# Autodesk Inventor assembly: WheelAssembly3.0
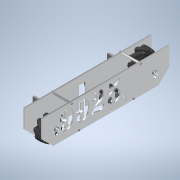
[picture p0: Inventor's stored thumbnail of the model, 180x180]
Saved by Autodesk Inventor 2021 (Build 250183000, 183)
## iProperties
Created: 2017-07-22
Part Number: WheelAssembly3.0
Document SubType Name: Assembly
Designer: User
Mass: 2301.48 g
Surface Area: 4071.67 cm^2
Volume: 902.346 cm^3
Density: 2.55055 g/cm^3
Author: User
## Documents named in this file (25)
- D:\robotics\CAD\2020-21-CAD\Drivetrain\drive train right.iam
- C:\Robotics\CAD\2016-17_CAD\Custom COTS\4inax.ipt
- C:\Robotics\CAD\2018-19_CAD\Offseason\InvertedDrivePlateOutside.ipt
- C:\Robotics\2018-19_CAD\Offseason\InvertedDrivePlateInside.ipt
- D:\robotics\CAD\COTSParts\Actobotics\535 parts\535198Bearing.25ID.5OD.ipt
- D:\robotics\CAD\COTSParts\Actobotics\Collar.ipt
- D:\robotics\CAD\COTSParts\Fasteners\6-32 SHCS x500.ipt
- D:\robotics\CAD\COTSParts\Fasteners\Hex Standoff 6-32 x2250.ipt
- D:\robotics\CAD\2020-21-CAD\Drivetrain\motor mount_MIR.ipt
- D:\robotics\CAD\COTSParts\Rev\REV-41-1657MecanumWheelRight.iam
- D:\robotics\CAD\2020-21-CAD\Drivetrain\motor mount.ipt
- D:\robotics\CAD\COTSParts\Tetrix\Tetrix hub - motor.ipt
- C:\Robotics\CAD\2016-17_CAD\Custom COTS\4inax_MIR1.ipt
- D:\robotics\CAD\COTSParts\Actobotics\535 parts\535198Bearing.25ID.5OD_MIR1.ipt
- D:\robotics\CAD\COTSParts\Actobotics\Collar_MIR1.ipt
- D:\robotics\CAD\COTSParts\Rev\REV-41-1657MecanumWheelRight_MIR.iam
- D:\robotics\CAD\COTSParts\Motors\am-3102NeveRest20 (1)_MIR_MIR.ipt
- D:\robotics\CAD\COTSParts\andymark\am-3902 am-3903 2in Omni 14mm Hex.ipt
- D:\robotics\CAD\COTSParts\Rev\REV-11-1271.STEP encoders.ipt
- D:\robotics\CAD\COTSParts\Actobotics\637 parts\637222 beval gear\615456 13tooth beval gear.ipt
- D:\robotics\CAD\COTSParts\Actobotics\637 parts\637222 beval gear\615460 26 tooth beval gear.ipt
- D:\robotics\CAD\COTSParts\Tetrix\Tetrix Hub - axle.ipt
- D:\robotics\CAD\COTSParts\Motors\am-3102NeveRest20 (1).ipt
- D:\robotics\CAD\2020-21-CAD\Drivetrain\InvertedDrivePlateInsideright.ipt
- D:\robotics\CAD\2020-21-CAD\Drivetrain\InvertedDrivePlateOutsideright.ipt
## Components (39 placed, 24 different names)
1. 4inax:4 — Insert:147, Mate:63, Mate:69
2. InvertedDrivePlateOutside:1 — Insert:71, Insert:128, Insert:129, Insert:130, Insert:131, Insert:136, Insert:137, Insert:138, Insert:139, Symmetry:1, Mate:80, Mate:84, Mate:86, Mate:91, Angle:3
3. InvertedDrivePlateInside:1 — Insert:90, Insert:132, Insert:133, Insert:134, Insert:135, Insert:140, Insert:141, Insert:142, Insert:143, Symmetry:1, Flush:10, Flush:11, Mate:73, Mate:82, Mate:83, Flush:13, Mate:85, Mate:97
4. 535198Bearing.25ID.5OD:1 — Insert:71, Insert:86
5. Collar:1 — Insert:86, Insert:147
6. 535198Bearing.25ID.5OD:5 — Insert:90
7. Hex Standoff 6-32 x2250:1 — Insert:129, Insert:134, Mate:108, Mate:117, Mate:118
8. Hex Standoff 6-32 x2250:2 — Insert:128, Insert:132, Mate:106, Mate:107, Mate:110, Mate:111
9. Hex Standoff 6-32 x2250:3 — Insert:131, Insert:135, Mate:115, Mate:116
10. Hex Standoff 6-32 x2250:4 — Insert:130, Insert:133, Mate:109, Mate:112, Mate:114
11. 6-32 SHCS x500:22 — Insert:136, Mate:123, Mate:124
12. 6-32 SHCS x500:23 — Insert:137, Mate:138, Mate:139
13. 6-32 SHCS x500:24 — Insert:138, Mate:125, Mate:126, Mate:127
14. 6-32 SHCS x500:25 — Insert:139, Mate:121, Mate:122
15. 6-32 SHCS x500:26 — Insert:140
16. 6-32 SHCS x500:27 — Insert:141, Mate:140, Mate:141
17. 6-32 SHCS x500:28 — Insert:142, Mate:119, Mate:120
18. 6-32 SHCS x500:29 — Insert:143, Mate:113
19. REV-41-1657MecanumWheelRight:1 [sub-assembly] — Mate:63, Mate:70, Mate:71, Mate:72, Flush:14, Mate:137
20. motor mount:1 — Flush:10, Flush:11, Mate:97, Mate:103, Flush:15, Flush:16, Flush:17, Mate:128, Mate:129, Mate:130
21. Tetrix hub - motor:1 — Mate:69, Mate:70, Mate:71, Mate:72, Mate:73, Mate:136
22. 4inax_MIR1:1 — Insert:150, Mate:76, Mate:80, Mate:92
23. 535198Bearing.25ID.5OD_MIR1:1 — Insert:151, Mate:84
24. Collar_MIR1:1 — Insert:150, Insert:151
25. 535198Bearing.25ID.5OD_MIR1:2 — Mate:82, Mate:83
26. REV-41-1657MecanumWheelRight_MIR:1 [sub-assembly] — Mate:76, Flush:14
27. motor mount_MIR:1 — Mate:78, Mate:79, Flush:13, Mate:85, Mate:95, Flush:16, Angle:4, Flush:17, Mate:131
28. am-3102NeveRest20 (1)_MIR_MIR:1 — Mate:78, Mate:79, Mate:96, Angle:4
29. am-3902 am-3903 2in Omni 14mm Hex:1 — Mate:89, Mate:90
30. REV-11-1271.STEP encoders:1 — Mate:86, Mate:89, Mate:90, Mate:91, Angle:3
31. 615456 13tooth beval gear:1 — Mate:92, Mate:105, Mate:132
32. 615460 26 tooth beval gear:1 — Mate:93, Mate:94, Mate:96, Mate:105
33. Tetrix Hub - axle:1 — Mate:93, Mate:94, Mate:95
34. 615460 26 tooth beval gear:2 — Mate:104, Mate:135
35. Tetrix Hub - axle:2
36. am-3102NeveRest20 (1):1 — Mate:103, Flush:15, Mate:104
37. InvertedDrivePlateInsideright:1 — Mate:110, Mate:111, Mate:113, Mate:114, Mate:115, Mate:117, Mate:119, Mate:120, Mate:128, Mate:129, Mate:130, Mate:131, Mate:132, Mate:133, Mate:134, Mate:140, Mate:141
38. InvertedDrivePlateOutsideright:1 — Mate:106, Mate:107, Mate:108, Mate:109, Mate:112, Mate:116, Mate:118, Mate:121, Mate:122, Mate:123, Mate:124, Mate:125, Mate:126, Mate:127, Mate:136, Mate:137, Mate:138, Mate:139
39. 615456 13tooth beval gear:2 — Mate:133, Mate:134, Mate:135
## Relationships (97: Mate 65, Insert 22, Flush 7, Angle 2, Symmetry 1)
- Insert:71: InvertedDrivePlateOutside:1 ↔ 535198Bearing.25ID.5OD:1
- Insert:86: 535198Bearing.25ID.5OD:1 ↔ Collar:1
- Insert:90: InvertedDrivePlateInside:1 ↔ 535198Bearing.25ID.5OD:5
- Insert:128: InvertedDrivePlateOutside:1 ↔ Hex Standoff 6-32 x2250:2
- Insert:129: InvertedDrivePlateOutside:1 ↔ Hex Standoff 6-32 x2250:1
- Insert:130: InvertedDrivePlateOutside:1 ↔ Hex Standoff 6-32 x2250:4
- Insert:131: InvertedDrivePlateOutside:1 ↔ Hex Standoff 6-32 x2250:3
- Insert:132: InvertedDrivePlateInside:1 ↔ Hex Standoff 6-32 x2250:2
- Insert:133: InvertedDrivePlateInside:1 ↔ Hex Standoff 6-32 x2250:4
- Insert:134: InvertedDrivePlateInside:1 ↔ Hex Standoff 6-32 x2250:1
- Insert:135: InvertedDrivePlateInside:1 ↔ Hex Standoff 6-32 x2250:3
- Insert:136: InvertedDrivePlateOutside:1 ↔ 6-32 SHCS x500:22
- Insert:137: InvertedDrivePlateOutside:1 ↔ 6-32 SHCS x500:23
- Insert:138: InvertedDrivePlateOutside:1 ↔ 6-32 SHCS x500:24
- Insert:139: InvertedDrivePlateOutside:1 ↔ 6-32 SHCS x500:25
- Insert:140: InvertedDrivePlateInside:1 ↔ 6-32 SHCS x500:26
- Insert:141: InvertedDrivePlateInside:1 ↔ 6-32 SHCS x500:27
- Insert:142: InvertedDrivePlateInside:1 ↔ 6-32 SHCS x500:28
- Insert:143: InvertedDrivePlateInside:1 ↔ 6-32 SHCS x500:29
- Insert:147: 4inax:4 ↔ Collar:1
- Symmetry:1: InvertedDrivePlateOutside:1 ↔ InvertedDrivePlateInside:1
- Mate:63: 4inax:4 ↔ REV-41-1657MecanumWheelRight:1
- Flush:10 (88.9 mm): InvertedDrivePlateInside:1 ↔ motor mount:1
- Flush:11 (-12.7 mm): InvertedDrivePlateInside:1 ↔ motor mount:1
- Mate:69: 4inax:4 ↔ Tetrix hub - motor:1
- Mate:70: REV-41-1657MecanumWheelRight:1 ↔ Tetrix hub - motor:1
- Mate:71: REV-41-1657MecanumWheelRight:1 ↔ Tetrix hub - motor:1
- Mate:72: REV-41-1657MecanumWheelRight:1 ↔ Tetrix hub - motor:1
- Mate:73 (19.05 mm): InvertedDrivePlateInside:1 ↔ Tetrix hub - motor:1
- Insert:150: 4inax_MIR1:1 ↔ Collar_MIR1:1
- Insert:151: 535198Bearing.25ID.5OD_MIR1:1 ↔ Collar_MIR1:1
- Mate:76: 4inax_MIR1:1 ↔ REV-41-1657MecanumWheelRight_MIR:1
- Mate:78: motor mount_MIR:1 ↔ am-3102NeveRest20 (1)_MIR_MIR:1
- Mate:79: motor mount_MIR:1 ↔ am-3102NeveRest20 (1)_MIR_MIR:1
- Mate:80: InvertedDrivePlateOutside:1 ↔ 4inax_MIR1:1
- Mate:82: InvertedDrivePlateInside:1 ↔ 535198Bearing.25ID.5OD_MIR1:2
- Mate:83: InvertedDrivePlateInside:1 ↔ 535198Bearing.25ID.5OD_MIR1:2
- Mate:84: InvertedDrivePlateOutside:1 ↔ 535198Bearing.25ID.5OD_MIR1:1
- Flush:13 (-88.9 mm): InvertedDrivePlateInside:1 ↔ motor mount_MIR:1
- Mate:85: InvertedDrivePlateInside:1 ↔ motor mount_MIR:1
- Flush:14: REV-41-1657MecanumWheelRight:1 ↔ REV-41-1657MecanumWheelRight_MIR:1
- Mate:86: InvertedDrivePlateOutside:1 ↔ REV-11-1271.STEP encoders:1
- Mate:89: am-3902 am-3903 2in Omni 14mm Hex:1 ↔ REV-11-1271.STEP encoders:1
- Mate:90: am-3902 am-3903 2in Omni 14mm Hex:1 ↔ REV-11-1271.STEP encoders:1
- Mate:91: InvertedDrivePlateOutside:1 ↔ REV-11-1271.STEP encoders:1
- Angle:3 (25 deg): InvertedDrivePlateOutside:1 ↔ REV-11-1271.STEP encoders:1
- Mate:92: 4inax_MIR1:1 ↔ 615456 13tooth beval gear:1
- Mate:93: 615460 26 tooth beval gear:1 ↔ Tetrix Hub - axle:1
- Mate:94: 615460 26 tooth beval gear:1 ↔ Tetrix Hub - axle:1
- Mate:95 (19.05 mm): motor mount_MIR:1 ↔ Tetrix Hub - axle:1
- Mate:96: am-3102NeveRest20 (1)_MIR_MIR:1 ↔ 615460 26 tooth beval gear:1
- Mate:97: InvertedDrivePlateInside:1 ↔ motor mount:1
- [Mate]: 615460 26 tooth beval gear:2 ↔ Tetrix Hub - axle:2
- [Mate]: 615460 26 tooth beval gear:2 ↔ Tetrix Hub - axle:2
- Mate:103: motor mount:1 ↔ am-3102NeveRest20 (1):1
- Flush:15: motor mount:1 ↔ am-3102NeveRest20 (1):1
- Mate:104: 615460 26 tooth beval gear:2 ↔ am-3102NeveRest20 (1):1
- Flush:16: motor mount:1 ↔ motor mount_MIR:1
- Angle:4 (17 deg): motor mount_MIR:1 ↔ am-3102NeveRest20 (1)_MIR_MIR:1
- Mate:105: 615456 13tooth beval gear:1 ↔ 615460 26 tooth beval gear:1
- Mate:106: Hex Standoff 6-32 x2250:2 ↔ InvertedDrivePlateOutsideright:1
- Mate:107: Hex Standoff 6-32 x2250:2 ↔ InvertedDrivePlateOutsideright:1
- Mate:108: Hex Standoff 6-32 x2250:1 ↔ InvertedDrivePlateOutsideright:1
- Mate:109: Hex Standoff 6-32 x2250:4 ↔ InvertedDrivePlateOutsideright:1
- Mate:110: Hex Standoff 6-32 x2250:2 ↔ InvertedDrivePlateInsideright:1
- Mate:111: Hex Standoff 6-32 x2250:2 ↔ InvertedDrivePlateInsideright:1
- Mate:112: Hex Standoff 6-32 x2250:4 ↔ InvertedDrivePlateOutsideright:1
- Mate:113: 6-32 SHCS x500:29 ↔ InvertedDrivePlateInsideright:1
- Mate:114: Hex Standoff 6-32 x2250:4 ↔ InvertedDrivePlateInsideright:1
- Mate:115: Hex Standoff 6-32 x2250:3 ↔ InvertedDrivePlateInsideright:1
- Mate:116: Hex Standoff 6-32 x2250:3 ↔ InvertedDrivePlateOutsideright:1
- Mate:117: Hex Standoff 6-32 x2250:1 ↔ InvertedDrivePlateInsideright:1
- Mate:118: Hex Standoff 6-32 x2250:1 ↔ InvertedDrivePlateOutsideright:1
- Mate:119: 6-32 SHCS x500:28 ↔ InvertedDrivePlateInsideright:1
- Mate:120: 6-32 SHCS x500:28 ↔ InvertedDrivePlateInsideright:1
- Mate:121: 6-32 SHCS x500:25 ↔ InvertedDrivePlateOutsideright:1
- Mate:122: 6-32 SHCS x500:25 ↔ InvertedDrivePlateOutsideright:1
- Mate:123: 6-32 SHCS x500:22 ↔ InvertedDrivePlateOutsideright:1
- Mate:124: 6-32 SHCS x500:22 ↔ InvertedDrivePlateOutsideright:1
- Mate:125: 6-32 SHCS x500:24 ↔ InvertedDrivePlateOutsideright:1
- Mate:126: 6-32 SHCS x500:24 ↔ InvertedDrivePlateOutsideright:1
- Mate:127: 6-32 SHCS x500:24 ↔ InvertedDrivePlateOutsideright:1
- Flush:17: motor mount:1 ↔ motor mount_MIR:1
- Mate:128: motor mount:1 ↔ InvertedDrivePlateInsideright:1
- Mate:129: motor mount:1 ↔ InvertedDrivePlateInsideright:1
- Mate:130: motor mount:1 ↔ InvertedDrivePlateInsideright:1
- Mate:131: motor mount_MIR:1 ↔ InvertedDrivePlateInsideright:1
- Mate:132: 615456 13tooth beval gear:1 ↔ InvertedDrivePlateInsideright:1
- Mate:133: InvertedDrivePlateInsideright:1 ↔ 615456 13tooth beval gear:2
- Mate:134: InvertedDrivePlateInsideright:1 ↔ 615456 13tooth beval gear:2
- Mate:135: 615460 26 tooth beval gear:2 ↔ 615456 13tooth beval gear:2
- Mate:136: Tetrix hub - motor:1 ↔ InvertedDrivePlateOutsideright:1
- Mate:137 (25.4 mm): REV-41-1657MecanumWheelRight:1 ↔ InvertedDrivePlateOutsideright:1
- Mate:138: 6-32 SHCS x500:23 ↔ InvertedDrivePlateOutsideright:1
- Mate:139: 6-32 SHCS x500:23 ↔ InvertedDrivePlateOutsideright:1
- Mate:140: 6-32 SHCS x500:27 ↔ InvertedDrivePlateInsideright:1
- Mate:141: 6-32 SHCS x500:27 ↔ InvertedDrivePlateInsideright:1
## Named parameters: d366_d360 = 0 mm, d367_d361 = 0 mm
